# Autodesk Inventor assembly: Pick_&_Place_Nozzle_Assembly
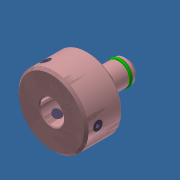
[picture p0: Inventor's stored thumbnail of the model, 180x180]
Saved by Autodesk Inventor 2015 (Build 190159000, 159)
## iProperties
Created: 2015-01-06
Part Number: Pick_&_Place_Nozzle_Assembly
Document SubType Name: Assembly
Designer: ice
Author: ice
## Documents named in this file (5)
- C:\Users\ice\Documents\GitHub\PnP-Magnetic-Tool-Tip\Inventor\Extender_Minimalist_Assembly.iam
- C:\Users\ice\Documents\GitHub\PnP-Magnetic-Tool-Tip\Inventor\o_ring_4.29_0.5.ipt
- C:\Users\ice\Documents\GitHub\PnP-Magnetic-Tool-Tip\Inventor\Extender_Minimalist.ipt
- C:\Users\ice\Documents\GitHub\PnP-Magnetic-Tool-Tip\Inventor\M2x5_Headless.ipt
- C:\Users\ice\Documents\GitHub\PnP-Magnetic-Tool-Tip\Inventor\Magnet10x1x5.ipt
## Components (7 placed, 4 different names)
1. Extender_Minimalist:1 — Mate:1, Mate:2, Flush:1, Flush:2, Mate:3, Mate:4, Mate:5, Mate:6, Mate:7, Mate:8, Mate:9, Flush:3
2. o_ring_4.29_0.5:1 — Mate:1, Flush:2
3. o_ring_4.29_0.5:2 — Mate:2, Flush:1
4. M2x5_Headless:1 — Mate:3, Mate:6
5. M2x5_Headless:2 — Mate:5, Mate:7
6. M2x5_Headless:3 — Mate:4, Mate:8
7. Magnet10x1x5:1 — Mate:9, Flush:3
## Relationships (12: Mate 9, Flush 3)
- Mate:1: Extender_Minimalist:1 ↔ o_ring_4.29_0.5:1
- Mate:2: Extender_Minimalist:1 ↔ o_ring_4.29_0.5:2
- Flush:1: Extender_Minimalist:1 ↔ o_ring_4.29_0.5:2
- Flush:2: Extender_Minimalist:1 ↔ o_ring_4.29_0.5:1
- Mate:3: Extender_Minimalist:1 ↔ M2x5_Headless:1
- Mate:4: Extender_Minimalist:1 ↔ M2x5_Headless:3
- Mate:5: Extender_Minimalist:1 ↔ M2x5_Headless:2
- Mate:6: Extender_Minimalist:1 ↔ M2x5_Headless:1
- Mate:7: Extender_Minimalist:1 ↔ M2x5_Headless:2
- Mate:8: Extender_Minimalist:1 ↔ M2x5_Headless:3
- Mate:9: Extender_Minimalist:1 ↔ Magnet10x1x5:1
- Flush:3: Extender_Minimalist:1 ↔ Magnet10x1x5:1
